# Autodesk Inventor assembly: case
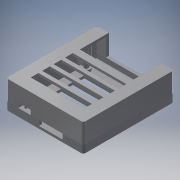
[picture p0: Inventor's stored thumbnail of the model, 180x180]
Saved by Autodesk Inventor 2018 (Build 220112000, 112)
## iProperties
Created: 2018-06-26
Part Number: case
Document SubType Name: Assembly
Designer: erwin
Author: erwin
## Documents named in this file (3)
- D:\GitHub\cloudberry-case\design\case.iam
- D:\GitHub\cloudberry-case\resources\Imported Components\orange_pi_r1_case_bottom\orange_pi_r1_case_bottom.ipt
- D:\GitHub\cloudberry-case\resources\Imported Components\orange_pi_r1_case_top\orange_pi_r1_case_top.ipt
## Components (2 placed, 2 different names)
1. orange_pi_r1_case_bottom:1 — Rigid:1
2. orange_pi_r1_case_top:1 — Rigid:1
## Relationships (1: WeldJoint 1)
- Rigid:1 [WeldJoint]: orange_pi_r1_case_bottom:1 ↔ orange_pi_r1_case_top:1
